# Autodesk Inventor assembly: useless machine
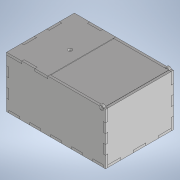
[picture p0: Inventor's stored thumbnail of the model, 180x180]
Saved by Autodesk Inventor 2020 (Build 240168000, 168)
## iProperties
Created: 2022-02-14
Part Number: useless machine
Document SubType Name: Assembly
Designer: rwte
Author: rwte
## Documents named in this file (6)
- C:\Users\chanc\Documents\GitHub\Dfab-AY21-22S2-Chan-Carl\CAD\final project\useless machine.iam
- C:\Users\chanc\Documents\GitHub\Dfab-AY21-22S2-Chan-Carl\CAD\final project\ipt files\arduino sitting.iam
- C:\Users\chanc\Documents\GitHub\Dfab-AY21-22S2-Chan-Carl\CAD\final project\ipt files\outer box.iam
- C:\Users\chanc\Documents\GitHub\Dfab-AY21-22S2-Chan-Carl\CAD\final project\ipt files\servo arm.ipt
- C:\Users\chanc\Documents\GitHub\Dfab-AY21-22S2-Chan-Carl\CAD\final project\ipt files\servo.ipt
- C:\Users\chanc\Documents\GitHub\Dfab-AY21-22S2-Chan-Carl\CAD\final project\ipt files\lid arm.ipt
## Components (5 placed, 5 different names)
1. arduino sitting:1 [sub-assembly] — Mate:1, Mate:2, Mate:3, Rotational:1, Mate:4
2. outer box:1 [sub-assembly] — Mate:1, Mate:2, Mate:3
3. servo arm:1 — Rotational:1
4. servo:1 — Mate:4, Rotational:2
5. lid arm:1 — Rotational:2
## Relationships (6: Mate 4, RevoluteJoint 2)
- Mate:1: arduino sitting:1 ↔ outer box:1
- Mate:2: arduino sitting:1 ↔ outer box:1
- Mate:3: arduino sitting:1 ↔ outer box:1
- Rotational:1 [RevoluteJoint]: arduino sitting:1 ↔ servo arm:1
- Mate:4: arduino sitting:1 ↔ servo:1
- Rotational:2 [RevoluteJoint]: servo:1 ↔ lid arm:1
